# Autodesk Inventor assembly: Ensamble Dispensador V2
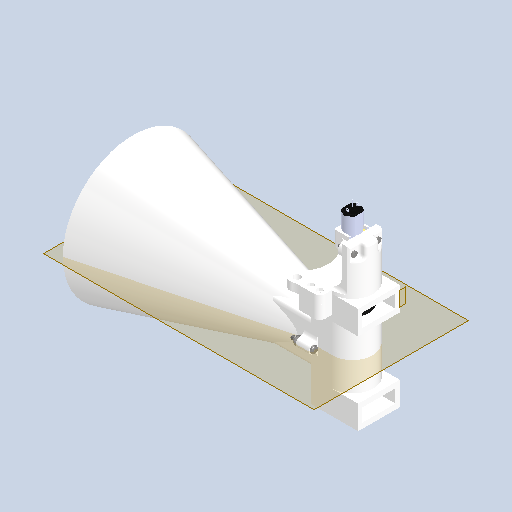
[picture p0: Inventor's stored thumbnail of the model, 512x512]
Saved by Autodesk Inventor 2022 (Build 260153000, 153)
## iProperties
Created: 2020-08-17
Part Number: Ensamble Dispensador V2
Document SubType Name: Assembly
Designer: juanp
Author: juanp
## Documents named in this file (10)
- C:\Users\juanp\OneDrive - Universidad de los andes\Uniandes\Robocol\EVA\V0  (Antiguo)\Dispensador V2\Ensamble Dispensador V2.iam
- C:\Users\juanp\OneDrive - Universidad de los andes\Uniandes\Robocol\EVA\V0  (Antiguo)\Dispensador V2\Tornillo.ipt
- C:\Users\juanp\OneDrive - Universidad de los andes\Uniandes\Robocol\EVA\V0  (Antiguo)\Dispensador V2\Tubo.ipt
- C:\Users\juanp\OneDrive - Universidad de los andes\Uniandes\Robocol\EVA\V0  (Antiguo)\Dispensador V2\Dud rodamiento.ipt
- C:\Users\juanp\Documents\Inventor\Content Center Files\R2020\en-US\ANSI B18.16.3M(2)\ANSI B18.16.3M - Property Class 5 and 10 - Metric M3 x 0.5 Metal Type.ipt
- C:\Users\juanp\Documents\Inventor\Content Center Files\R2020\en-US\ANSI B18.3.4M(1)\ANSI B18.3.4M - M3 x 0.5 x 16(2).ipt
- C:\Users\juanp\OneDrive - Universidad de los andes\Uniandes\Robocol\EVA\V0  (Antiguo)\Motor\micro-metal-gearmotor-extended-with-1086-bracket.ipt
- C:\Users\juanp\OneDrive - Universidad de los andes\Uniandes\Robocol\EVA\V0  (Antiguo)\Dispensador V2\Acoplador Eje.ipt
- C:\Users\juanp\Documents\Inventor\Content Center Files\R2020\en-US\ANSI B18.6.3(03)\ANSI B18.6.3 - 2-64 UNF - 0.4375(14).ipt
- C:\Users\juanp\Documents\Inventor\Content Center Files\R2020\en-US\ANSI B 18.2.4.1 M(1)\ANSI B 18.2.4.1 M - M2.5 x 0.45Style 1.ipt
## Components (14 placed, 9 different names)
1. Tornillo:1 — Mate:1, Mate:2, Mate:17
2. Tubo:1 — Mate:1, Mate:2, Flush:1, Mate:3, Mate:6, Flush:2, Mate:11, Mate:12, Mate:13, Mate:16, Mate:18, Mate:20, Mate:21, Mate:24, Mate:26, Mate:31, Mate:33, Mate:34, Mate:35
3. Dud rodamiento:1 — Flush:1, Mate:3
4. Dud rodamiento:2 — Mate:6, Flush:2
5. Prevailing Torque Type Hex Nut - Steel Metric Property Class 5 and 10 - Metric M3 x 0.5 Metal Type:2 — Mate:23, Mate:24
6. Broached Hexagon Socket Button Head Cap Screw - Metric M3 x 0.5 x 16:1 — Mate:11, Mate:12, Mate:23
7. Prevailing Torque Type Hex Nut - Steel Metric Property Class 5 and 10 - Metric M3 x 0.5 Metal Type:3 — Mate:25, Mate:26
8. Broached Hexagon Socket Button Head Cap Screw - Metric M3 x 0.5 x 16:2 — Mate:13, Mate:16, Mate:25
9. micro-metal-gearmotor-extended-with-1086-bracket:1 — Mate:19, Mate:20, Mate:21, Mate:27, Mate:28, Mate:29, Mate:30, Angle:1, Angle:2
10. Acoplador Eje:1 — Mate:17, Mate:18, Mate:19
11. Cross Recessed Binding Head Machine Screw - Type I - Inch No. 2 - 64 - 7/16:1 — Mate:33, Mate:35
12. Cross Recessed Binding Head Machine Screw - Type I - Inch No. 2 - 64 - 7/16:2 — Mate:31, Mate:34
13. Hex Nut Metric M2.5 x 0.45:1 — Mate:27, Mate:30, Angle:2
14. Hex Nut Metric M2.5 x 0.45:2 — Mate:28, Mate:29, Angle:1
## Relationships (29: Mate 25, Flush 2, Angle 2)
- Mate:1: Tornillo:1 ↔ Tubo:1
- Mate:2: Tornillo:1 ↔ Tubo:1
- Flush:1: Tubo:1 ↔ Dud rodamiento:1
- Mate:3: Tubo:1 ↔ Dud rodamiento:1
- Mate:6: Tubo:1 ↔ Dud rodamiento:2
- Flush:2: Tubo:1 ↔ Dud rodamiento:2
- Mate:11: Tubo:1 ↔ Broached Hexagon Socket Button Head Cap Screw - Metric M3 x 0.5 x 16:1
- Mate:12: Tubo:1 ↔ Broached Hexagon Socket Button Head Cap Screw - Metric M3 x 0.5 x 16:1
- Mate:13: Tubo:1 ↔ Broached Hexagon Socket Button Head Cap Screw - Metric M3 x 0.5 x 16:2
- Mate:16: Tubo:1 ↔ Broached Hexagon Socket Button Head Cap Screw - Metric M3 x 0.5 x 16:2
- Mate:17: Tornillo:1 ↔ Acoplador Eje:1
- Mate:18: Tubo:1 ↔ Acoplador Eje:1
- Mate:19: micro-metal-gearmotor-extended-with-1086-bracket:1 ↔ Acoplador Eje:1
- Mate:20: Tubo:1 ↔ micro-metal-gearmotor-extended-with-1086-bracket:1
- Mate:21: Tubo:1 ↔ micro-metal-gearmotor-extended-with-1086-bracket:1
- Mate:23: Prevailing Torque Type Hex Nut - Steel Metric Property Class 5 and 10 - Metric M3 x 0.5 Metal Type:2 ↔ Broached Hexagon Socket Button Head Cap Screw - Metric M3 x 0.5 x 16:1
- Mate:24: Tubo:1 ↔ Prevailing Torque Type Hex Nut - Steel Metric Property Class 5 and 10 - Metric M3 x 0.5 Metal Type:2
- Mate:25: Prevailing Torque Type Hex Nut - Steel Metric Property Class 5 and 10 - Metric M3 x 0.5 Metal Type:3 ↔ Broached Hexagon Socket Button Head Cap Screw - Metric M3 x 0.5 x 16:2
- Mate:26: Tubo:1 ↔ Prevailing Torque Type Hex Nut - Steel Metric Property Class 5 and 10 - Metric M3 x 0.5 Metal Type:3
- Mate:27: micro-metal-gearmotor-extended-with-1086-bracket:1 ↔ Hex Nut Metric M2.5 x 0.45:1
- Mate:28: micro-metal-gearmotor-extended-with-1086-bracket:1 ↔ Hex Nut Metric M2.5 x 0.45:2
- Mate:29: micro-metal-gearmotor-extended-with-1086-bracket:1 ↔ Hex Nut Metric M2.5 x 0.45:2
- Mate:30: micro-metal-gearmotor-extended-with-1086-bracket:1 ↔ Hex Nut Metric M2.5 x 0.45:1
- Angle:1 (0 deg): micro-metal-gearmotor-extended-with-1086-bracket:1 ↔ Hex Nut Metric M2.5 x 0.45:2
- Angle:2 (0 deg): micro-metal-gearmotor-extended-with-1086-bracket:1 ↔ Hex Nut Metric M2.5 x 0.45:1
- Mate:31: Tubo:1 ↔ Cross Recessed Binding Head Machine Screw - Type I - Inch No. 2 - 64 - 7/16:2
- Mate:33: Tubo:1 ↔ Cross Recessed Binding Head Machine Screw - Type I - Inch No. 2 - 64 - 7/16:1
- Mate:34: Tubo:1 ↔ Cross Recessed Binding Head Machine Screw - Type I - Inch No. 2 - 64 - 7/16:2
- Mate:35: Tubo:1 ↔ Cross Recessed Binding Head Machine Screw - Type I - Inch No. 2 - 64 - 7/16:1
